# Autodesk Inventor assembly: front-mechanizm
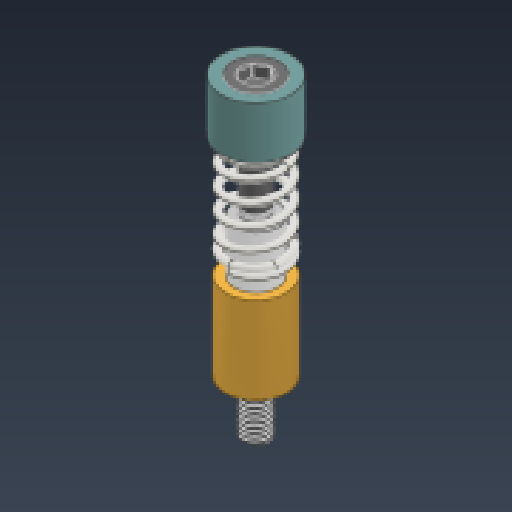
[picture p0: Inventor's stored thumbnail of the model, 512x512]
Saved by Autodesk Inventor 2023 (Build 270158000, 158)
## iProperties
Created: 2025-03-30
Part Number: front-mechanizm
Document SubType Name: Assembly
Designer: szymo
Mass: 6 g
Surface Area: 18.8088 cm^2
Volume: 0.912994 cm^3
Density: 6.57178 g/cm^3
Author: szymo
## Documents named in this file (6)
- D:\tech\robotyka\robots\evangelion\inventor-project\front-mechanizm.iam
- D:\tech\robotyka\robots\evangelion\inventor-project\rod.ipt
- D:\tech\robotyka\robots\evangelion\inventor-project\Compress Spring11.ipt
- D:\tech\robotyka\robots\evangelion\inventor-project\rozszerzenie-m3.ipt
- D:\tech\robotyka\robots\evangelion\inventor-project\lozysko sf-1.ipt
- D:\tech\robotyka\robots\evangelion\inventor-project\screws\m3x20M3.ipt
## Components (6 placed, 6 different names)
1. rod:1 — Mate:8, Flush:1, Mate:12, Mate:15, Mate:16, Mate:17
2. Compress Spring1:1 — Mate:11, Mate:17
3. lozysko sf-1:1 — Mate:8, Flush:1, Flush:18
4. rozszerzenie-m3:1 — Mate:11, Mate:13, Mate:14, Flush:18
5. m3x20:1 — Mate:12, Mate:13, Mate:14
6. m3x20M3:2 — Mate:15, Mate:16
## Relationships (10: Mate 8, Flush 2)
- Mate:8: rod:1 ↔ lozysko sf-1:1
- Flush:1: rod:1 ↔ lozysko sf-1:1
- Mate:11: Compress Spring1:1 ↔ rozszerzenie-m3:1
- Mate:12: rod:1 ↔ m3x20:1
- Mate:13: rozszerzenie-m3:1 ↔ m3x20:1
- Mate:14: rozszerzenie-m3:1 ↔ m3x20:1
- Mate:15: rod:1 ↔ m3x20M3:2
- Mate:16: rod:1 ↔ m3x20M3:2
- Flush:18 (-20 mm): lozysko sf-1:1 ↔ rozszerzenie-m3:1
- Mate:17: rod:1 ↔ Compress Spring1:1
